# Autodesk Inventor assembly: OBG-Grundplatte
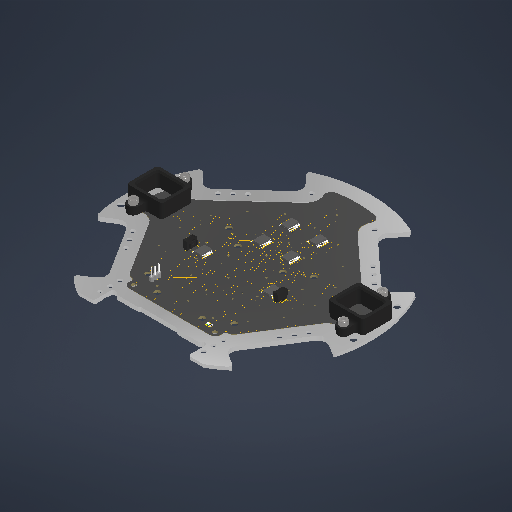
[picture p0: Inventor's stored thumbnail of the model, 512x512]
Saved by Autodesk Inventor 2025.2 (Build 292293000, 293)
## iProperties
Created: 2024-11-26
Part Number: OBG-Grundplatte
Document SubType Name: Assembly
Designer: Fabian
Author: Fabian
## Documents named in this file (6)
- C:\Users\Faabs\Desktop\HBG v2025\Oberbaugruppen\OBG-Grundplatte\OBG-Grundplatte.iam
- C:\Users\Faabs\Desktop\HBG v2025\Oberbaugruppen\OBG-Grundplatte\Bauteile\Grundplatte.ipt
- C:\Users\Faabs\Desktop\HBG v2025\Oberbaugruppen\OBG-Grundplatte\Bauteile\Bodenplatine.iam
- C:\Users\Faabs\Desktop\HBG v2025\Oberbaugruppen\OBG-Grundplatte\Bauteile\SchussAkkuHalterung.ipt
- C:\Users\Faabs\Desktop\HBG v2025\Oberbaugruppen\OBG-Grundplatte\Bauteile\SchussAkkuHalterung_MIR.ipt
- C:\Users\Faabs\Desktop\HBG v2025\Verbindungselemente\DIN 912\DIN 912 - M3 x 0,5 x 8 x 6,75.ipt
## Components (8 placed, 5 different names)
1. Bodenplatine:1 [sub-assembly] — Passend:5, Passend:6, Fluchtend:1
2. Grundplatte:1 — Passend:1, Passend:2, Passend:3, Passend:5, Passend:6, Passend:10, Passend:11, Passend:12, Passend:13, Passend:14, Passend:15, Fluchtend:1
3. SchussAkkuHalterung:1 — Einfügen:1, Einfügen:2, Passend:13, Passend:14, Passend:15
4. SchussAkkuHalterung_MIR:1 — Passend:10, Passend:11, Passend:12, Einfügen:3, Einfügen:4
5. DIN 912 - ersetzt durch DIN EN ISO 4762 M3 x 8:1 — Einfügen:3
6. DIN 912 - ersetzt durch DIN EN ISO 4762 M3 x 8:2 — Einfügen:4
7. DIN 912 - ersetzt durch DIN EN ISO 4762 M3 x 8:3 — Einfügen:1
8. DIN 912 - ersetzt durch DIN EN ISO 4762 M3 x 8:4 — Einfügen:2
## Relationships (16: Mate 11, Insert 4, Flush 1)
- Passend:1 [Mate]: Grundplatte:1
- Passend:2 [Mate]: Grundplatte:1
- Passend:3 [Mate]: Grundplatte:1
- Passend:5 [Mate]: Bodenplatine:1 ↔ Grundplatte:1
- Passend:6 [Mate]: Bodenplatine:1 ↔ Grundplatte:1
- Passend:10 [Mate]: Grundplatte:1 ↔ SchussAkkuHalterung_MIR:1
- Passend:11 [Mate]: Grundplatte:1 ↔ SchussAkkuHalterung_MIR:1
- Passend:12 [Mate]: Grundplatte:1 ↔ SchussAkkuHalterung_MIR:1
- Einfügen:1 [Insert]: SchussAkkuHalterung:1 ↔ DIN 912 - ersetzt durch DIN EN ISO 4762 M3 x 8:3
- Einfügen:2 [Insert]: SchussAkkuHalterung:1 ↔ DIN 912 - ersetzt durch DIN EN ISO 4762 M3 x 8:4
- Einfügen:3 [Insert]: SchussAkkuHalterung_MIR:1 ↔ DIN 912 - ersetzt durch DIN EN ISO 4762 M3 x 8:1
- Einfügen:4 [Insert]: SchussAkkuHalterung_MIR:1 ↔ DIN 912 - ersetzt durch DIN EN ISO 4762 M3 x 8:2
- Passend:13 [Mate]: Grundplatte:1 ↔ SchussAkkuHalterung:1
- Passend:14 [Mate]: Grundplatte:1 ↔ SchussAkkuHalterung:1
- Passend:15 [Mate]: Grundplatte:1 ↔ SchussAkkuHalterung:1
- Fluchtend:1 [Flush]: Bodenplatine:1 ↔ Grundplatte:1
